# Autodesk Inventor assembly: Assembly1
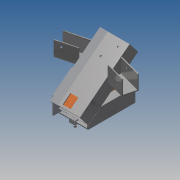
[picture p0: Inventor's stored thumbnail of the model, 180x180]
Saved by Autodesk Inventor 2014 SP1 (Build 180222100, 222)
## iProperties
Created: 2015-03-20
Part Number: Assembly1
Document SubType Name: Assembly
Designer: ddeboer
Author: ddeboer
## Documents named in this file (3)
- C:\Users\Dave\Desktop\hera-cad\endcaps\compare.iam
- C:\Users\Dave\Desktop\hera-cad\support\endAssembly.iam
- C:\Users\Dave\Desktop\hera-cad\endcaps\fabrication model end cap left.iam
## Components (2 placed, 2 different names)
1. endAssembly:1 [sub-assembly] — Flush:1, Flush:2, Flush:3
2. fabrication model end cap left:1 [sub-assembly] — Flush:1, Flush:2, Flush:3
## Relationships (3: Flush 3)
- Flush:1: endAssembly:1 ↔ fabrication model end cap left:1
- Flush:2: endAssembly:1 ↔ fabrication model end cap left:1
- Flush:3: endAssembly:1 ↔ fabrication model end cap left:1
